# Autodesk Inventor assembly: CAM_Assembly
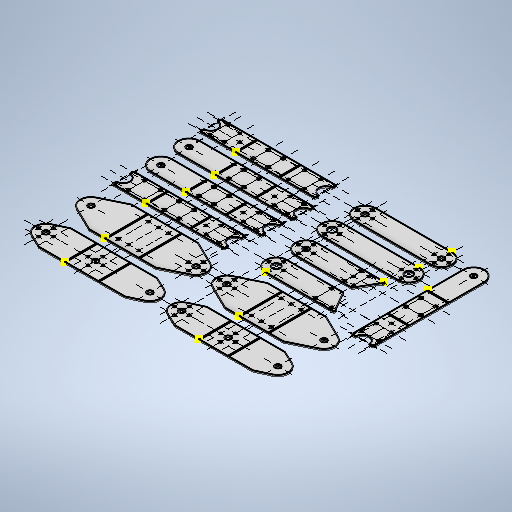
[picture p0: Inventor's stored thumbnail of the model, 512x512]
Saved by Autodesk Inventor 2026.1 (Build 301233000, 233)
## iProperties
Created: 2025-08-09
Part Number: CAM_Assembly
Document SubType Name: Assembly
Designer: User
Author: User
## Documents named in this file (13)
- C:\Users\User\Documents\The Maverick's Files\College 3-3\로보인 프로젝트\RHp_Humanoid_ver1\CAM\CAM_T1.5.iam
- C:\Users\User\Documents\The Maverick's Files\College 3-3\로보인 프로젝트\RHp_Humanoid_ver1\CAM\CAM_axis_1_top_frame.ipt
- C:\Users\User\Documents\The Maverick's Files\College 3-3\로보인 프로젝트\RHp_Humanoid_ver1\CAM\CAM_axis_1_supplement_frame.ipt
- C:\Users\User\Documents\The Maverick's Files\College 3-3\로보인 프로젝트\RHp_Humanoid_ver1\CAM\CAM_axis_2_4_connector_frame_non_powered.ipt
- C:\Users\User\Documents\The Maverick's Files\College 3-3\로보인 프로젝트\RHp_Humanoid_ver1\CAM\CAM_axis_2_4_connector_frame_powered.ipt
- C:\Users\User\Documents\The Maverick's Files\College 3-3\로보인 프로젝트\RHp_Humanoid_ver1\CAM\CAM_axis_2_bottom_frame.ipt
- C:\Users\User\Documents\The Maverick's Files\College 3-3\로보인 프로젝트\RHp_Humanoid_ver1\CAM\CAM_axis_3_bottom_frame.ipt
- C:\Users\User\Documents\The Maverick's Files\College 3-3\로보인 프로젝트\RHp_Humanoid_ver1\CAM\CAM_axis_4_5_connector_frame_non_powered.ipt
- C:\Users\User\Documents\The Maverick's Files\College 3-3\로보인 프로젝트\RHp_Humanoid_ver1\CAM\CAM_axis_4_5_connector_frame_powered.ipt
- C:\Users\User\Documents\The Maverick's Files\College 3-3\로보인 프로젝트\RHp_Humanoid_ver1\CAM\CAM_axis_5_top_frame.ipt
- C:\Users\User\Documents\The Maverick's Files\College 3-3\로보인 프로젝트\RHp_Humanoid_ver1\CAM\CAM_axis_6_bottom_frame(top).ipt
- C:\Users\User\Documents\The Maverick's Files\College 3-3\로보인 프로젝트\RHp_Humanoid_ver1\CAM\CAM_axis_6_supplement_frame.ipt
- C:\Users\User\Documents\The Maverick's Files\College 3-3\로보인 프로젝트\RHp_Humanoid_ver1\CAM\CAM_axis_6_top_frame.ipt
## Components (13 placed, 12 different names)
1. CAM_axis_1_top_frame:1 — Flush:1, Flush:2, Flush:3, Flush:4, Flush:5, Flush:6, Flush:7, Flush:8, Flush:9, Flush:10, Flush:11, Mate:6, Flush:17, Mate:22, Mate:23, Mate:24
2. CAM_axis_1_supplement_frame:1 — Flush:4, Flush:17, Mate:22, Mate:25, Mate:26
3. CAM_axis_2_4_connector_frame_non_powered:1 — Flush:16, Mate:17, Mate:21, Flush:19
4. CAM_axis_2_4_connector_frame_powered:1 — Flush:7, Flush:15, Flush:16, Mate:16, Mate:17, Mate:19, Flush:18
5. CAM_axis_2_bottom_frame:1 — Mate:3, Flush:5, Mate:14, Mate:21, Mate:27, Mate:28, Mate:29
6. CAM_axis_3_bottom_frame:1 — Mate:3, Flush:6, Mate:6, Mate:11, Mate:12, Mate:19
7. CAM_axis_4_5_connector_frame_non_powered:1 — Flush:14, Flush:15, Mate:15, Mate:16, Mate:20
8. CAM_axis_4_5_connector_frame_powered:1 — Flush:12, Flush:13, Flush:14, Mate:15, Mate:18
9. CAM_axis_5_top_frame:1 — Flush:10, Mate:13, Mate:14, Flush:12, Flush:13, Mate:18
10. CAM_axis_6_bottom_frame(top):1 — Flush:9, Mate:23, Mate:24, Mate:27, Mate:28
11. CAM_axis_6_supplement_frame:1 — Flush:8, Mate:25, Mate:26
12. CAM_axis_6_top_frame:1 — Flush:11, Mate:11, Mate:12, Mate:13, Mate:20
13. CAM_axis_3_bottom_frame:2 — Mate:29, Flush:18, Flush:19
## Relationships (40: Mate 21, Flush 19)
- Flush:1: CAM_axis_1_top_frame:1
- Flush:2: CAM_axis_1_top_frame:1
- Flush:3: CAM_axis_1_top_frame:1
- Mate:3 (8 mm): CAM_axis_2_bottom_frame:1 ↔ CAM_axis_3_bottom_frame:1
- Flush:4: CAM_axis_1_top_frame:1 ↔ CAM_axis_1_supplement_frame:1
- Flush:5: CAM_axis_1_top_frame:1 ↔ CAM_axis_2_bottom_frame:1
- Flush:6: CAM_axis_1_top_frame:1 ↔ CAM_axis_3_bottom_frame:1
- Mate:6: CAM_axis_1_top_frame:1 ↔ CAM_axis_3_bottom_frame:1
- Flush:7: CAM_axis_1_top_frame:1 ↔ CAM_axis_2_4_connector_frame_powered:1
- Flush:8: CAM_axis_1_top_frame:1 ↔ CAM_axis_6_supplement_frame:1
- Flush:9: CAM_axis_1_top_frame:1 ↔ CAM_axis_6_bottom_frame(top):1
- Flush:10: CAM_axis_1_top_frame:1 ↔ CAM_axis_5_top_frame:1
- Flush:11: CAM_axis_1_top_frame:1 ↔ CAM_axis_6_top_frame:1
- Mate:11 (8 mm): CAM_axis_3_bottom_frame:1 ↔ CAM_axis_6_top_frame:1
- Mate:12: CAM_axis_3_bottom_frame:1 ↔ CAM_axis_6_top_frame:1
- Mate:13 (8 mm): CAM_axis_5_top_frame:1 ↔ CAM_axis_6_top_frame:1
- Mate:14: CAM_axis_2_bottom_frame:1 ↔ CAM_axis_5_top_frame:1
- Flush:12: CAM_axis_4_5_connector_frame_powered:1 ↔ CAM_axis_5_top_frame:1
- Flush:13: CAM_axis_4_5_connector_frame_powered:1 ↔ CAM_axis_5_top_frame:1
- Flush:14: CAM_axis_4_5_connector_frame_non_powered:1 ↔ CAM_axis_4_5_connector_frame_powered:1
- Flush:15: CAM_axis_2_4_connector_frame_powered:1 ↔ CAM_axis_4_5_connector_frame_non_powered:1
- Flush:16: CAM_axis_2_4_connector_frame_non_powered:1 ↔ CAM_axis_2_4_connector_frame_powered:1
- Mate:15 (8 mm): CAM_axis_4_5_connector_frame_non_powered:1 ↔ CAM_axis_4_5_connector_frame_powered:1
- Mate:16 (8 mm): CAM_axis_2_4_connector_frame_powered:1 ↔ CAM_axis_4_5_connector_frame_non_powered:1
- Mate:17 (8 mm): CAM_axis_2_4_connector_frame_non_powered:1 ↔ CAM_axis_2_4_connector_frame_powered:1
- Mate:18 (30 mm): CAM_axis_4_5_connector_frame_powered:1 ↔ CAM_axis_5_top_frame:1
- Mate:19 (-25 mm): CAM_axis_2_4_connector_frame_powered:1 ↔ CAM_axis_3_bottom_frame:1
- Mate:20 (20 mm): CAM_axis_4_5_connector_frame_non_powered:1 ↔ CAM_axis_6_top_frame:1
- Mate:21 (32 mm): CAM_axis_2_4_connector_frame_non_powered:1 ↔ CAM_axis_2_bottom_frame:1
- Flush:17: CAM_axis_1_top_frame:1 ↔ CAM_axis_1_supplement_frame:1
- Mate:22 (30 mm): CAM_axis_1_top_frame:1 ↔ CAM_axis_1_supplement_frame:1
- Mate:23: CAM_axis_1_top_frame:1 ↔ CAM_axis_6_bottom_frame(top):1
- Mate:24 (8 mm): CAM_axis_1_top_frame:1 ↔ CAM_axis_6_bottom_frame(top):1
- Mate:25: CAM_axis_1_supplement_frame:1 ↔ CAM_axis_6_supplement_frame:1
- Mate:26 (8 mm): CAM_axis_1_supplement_frame:1 ↔ CAM_axis_6_supplement_frame:1
- Mate:27 (8 mm): CAM_axis_2_bottom_frame:1 ↔ CAM_axis_6_bottom_frame(top):1
- Mate:28: CAM_axis_2_bottom_frame:1 ↔ CAM_axis_6_bottom_frame(top):1
- Mate:29 (130 mm): CAM_axis_2_bottom_frame:1 ↔ CAM_axis_3_bottom_frame:2
- Flush:18: CAM_axis_2_4_connector_frame_powered:1 ↔ CAM_axis_3_bottom_frame:2
- Flush:19 (10 mm): CAM_axis_2_4_connector_frame_non_powered:1 ↔ CAM_axis_3_bottom_frame:2
